# Autodesk Inventor assembly: Victor884
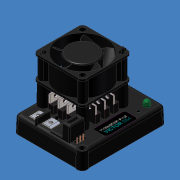
[picture p0: Inventor's stored thumbnail of the model, 180x180]
Saved by Autodesk Inventor 2011 SP1 (Build 150282100, 282)
## iProperties
Shininess: 64.0
Length Units: 11272
Angle Units: 11279
Time Units: 11290
Mass Units: 11286
Length Display Precision: 3
Angle Display Precision: 2
Compacted: True
Part Number: Victor884
Document SubType Name: Assembly
Created: 2007-01-15
Designer: uidk0133
Density: 0.0
Volumn: 0.0
Area: 0.0
PropertySet Name: Model Information
Control State: 0
Master: False
Checked Out: False
Author: uidk0133
## Documents named in this file (9)
- C:\Dropbox\Autobot\Design\Library\Victor884\Victor884.iam
- C:\Dropbox\Autobot\Design\Library\Victor884\Victor884-Cover.ipt
- C:\Dropbox\Autobot\Design\Library\Victor884\Fan-PAPST-412.ipt
- C:\Dropbox\Autobot\Design\Library\Victor884\Victor884-Base.ipt
- C:\Dropbox\Autobot\Design\Library\Victor884\Victor884-Capacitor.ipt
- C:\Dropbox\Autobot\Design\Library\Victor884\Victor884-LED - Green.ipt
- C:\Dropbox\Autobot\Design\Library\Victor884\Victor884-Fet.ipt
- C:\Dropbox\Autobot\Design\Library\Victor884\Victor884 Screw Terminal.ipt
- C:\Dropbox\Autobot\Design\Library\Victor884\Victor884-3 Pin Connector.ipt
## Components (22 placed, 8 different names)
1. Victor884-Cover:1 — Mate:1, Mate:2, Mate:3, Mate:4, Mate:5, Angle:1, Mate:6, Mate:7, Mate:8, Mate:9, Flush:2, Flush:3, Flush:4, Flush:9, Flush:13, Mate:12
2. Fan-PAPST-412:1 — Mate:4, Mate:5, Angle:1, Flush:1, Flush:10, Mate:10, Mate:13, Mate:14
3. Victor884-Base:1 — Mate:1, Mate:2, Mate:3
4. Victor884-Capacitor:1 — Mate:6, Flush:13
5. Victor884-LED - Green:1 — Mate:7, Mate:8
6. Victor884-3 Pin Connector:1 — Mate:12, Mate:13, Mate:14
7. Victor884-Fet:3 — Flush:3, Flush:6, Flush:8
8. Victor884-Fet:2 — Flush:4, Flush:5, Flush:7, Flush:8
9. Victor884-Fet:1 — Mate:9, Flush:1, Flush:2, Flush:5, Flush:6, Flush:7
10. Victor884-Fet:4
11. Victor884-Fet:5
12. Victor884-Fet:6
13. Victor884-Fet:7
14. Victor884-Fet:8
15. Victor884-Fet:9
16. Victor884-Fet:10
17. Victor884-Fet:11
18. Victor884-Fet:12
19. Victor884 Screw Terminal:1 — Flush:9, Flush:10, Mate:10, Flush:11, Flush:12, Mate:11
20. Victor884 Screw Terminal:2 — Flush:11, Flush:12, Mate:11
21. Victor884 Screw Terminal:3
22. Victor884 Screw Terminal:4
## Component patterns: (4 elements, first: Victor884-Fet:3 + Victor884-Fet:2 + Victor884-Fet:1), (2 elements, first: Victor884 Screw Terminal:1 + Victor884 Screw Terminal:2)
## Relationships (28: Mate 14, Flush 13, Angle 1)
- Mate:1: Victor884-Cover:1 ↔ Victor884-Base:1
- Mate:2: Victor884-Cover:1 ↔ Victor884-Base:1
- Mate:3: Victor884-Cover:1 ↔ Victor884-Base:1
- Mate:4: Victor884-Cover:1 ↔ Fan-PAPST-412:1
- Mate:5: Victor884-Cover:1 ↔ Fan-PAPST-412:1
- Angle:1 (0 deg): Victor884-Cover:1 ↔ Fan-PAPST-412:1
- Mate:6: Victor884-Cover:1 ↔ Victor884-Capacitor:1
- Mate:7: Victor884-Cover:1 ↔ Victor884-LED - Green:1
- Mate:8 (1.27 mm): Victor884-Cover:1 ↔ Victor884-LED - Green:1
- Mate:9 (0.254 mm): Victor884-Cover:1 ↔ Victor884-Fet:1
- Flush:1 (1.016 mm): Fan-PAPST-412:1 ↔ Victor884-Fet:1
- Flush:2: Victor884-Cover:1 ↔ Victor884-Fet:1
- Flush:3: Victor884-Cover:1 ↔ Victor884-Fet:3
- Flush:4: Victor884-Cover:1 ↔ Victor884-Fet:2
- Flush:5: Victor884-Fet:2 ↔ Victor884-Fet:1
- Flush:6: Victor884-Fet:3 ↔ Victor884-Fet:1
- Flush:7 (-7.366 mm): Victor884-Fet:2 ↔ Victor884-Fet:1
- Flush:8 (-7.366 mm): Victor884-Fet:3 ↔ Victor884-Fet:2
- Flush:9 (-0.762 mm): Victor884-Cover:1 ↔ Victor884 Screw Terminal:1
- Flush:10 (-5.969 mm): Fan-PAPST-412:1 ↔ Victor884 Screw Terminal:1
- Mate:10 (2.032 mm): Fan-PAPST-412:1 ↔ Victor884 Screw Terminal:1
- Flush:11: Victor884 Screw Terminal:1 ↔ Victor884 Screw Terminal:2
- Flush:12: Victor884 Screw Terminal:1 ↔ Victor884 Screw Terminal:2
- Mate:11 (10.16 mm): Victor884 Screw Terminal:1 ↔ Victor884 Screw Terminal:2
- Flush:13 (15.24 mm): Victor884-Cover:1 ↔ Victor884-Capacitor:1
- Mate:12: Victor884-Cover:1 ↔ Victor884-3 Pin Connector:1
- Mate:13 (3.683 mm): Fan-PAPST-412:1 ↔ Victor884-3 Pin Connector:1
- Mate:14 (2.032 mm): Fan-PAPST-412:1 ↔ Victor884-3 Pin Connector:1
